# Autodesk Inventor assembly: 200-40-BOGIE-CONNECTOR-ASM-01
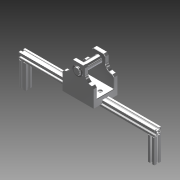
[picture p0: Inventor's stored thumbnail of the model, 180x180]
Saved by Autodesk Inventor 2018.2 (Build 222227000, 227)
## iProperties
Manager: feesmrt
Company: FRANC0R
Created: 2017-12-10
Part Number: 200-40-BOGIE-CONNECTOR-ASM-01
Material: Generisch
Document SubType Name: Assembly
Designer: feesmrt
Project: Rescue Robot
Cost Center: -
Description: Bogie Connector Assembly
Engineer: feesmrt
Authority: feesmrt
Stock Number: 200-40-BOGIE-CONNECTOR-ASM-01
Author: feesmrt
Title: Bogie Connector Assembly
Subject: Rescue Robot
Revision Number: 1
## Documents named in this file (6)
- D:\Programmierung\FRANC0R\CAD\02-Rocker-Bogie-Robot\200-ROCKER-BOGIE\200-40-BOGIE-CONNECTOR-ASM-01.iam
- D:\Programmierung\FRANC0R\CAD\02-Rocker-Bogie-Robot\200-ROCKER-BOGIE\200-40-BOGIE-CONNECTOR-01.ipt
- D:\Programmierung\FRANC0R\CAD\02-Rocker-Bogie-Robot\200-ROCKER-BOGIE\200-40-BOGIE-CONNECTOR-02.ipt
- D:\Programmierung\FRANC0R\CAD\02-Rocker-Bogie-Robot\900-COMPONENTS\900-50-PROFILES\90-50-PROFILES-20x20x400.ipt
- D:\Programmierung\FRANC0R\CAD\02-Rocker-Bogie-Robot\900-COMPONENTS\900-50-PROFILES\90-50-PROFILES-20x20x70.ipt
- D:\Programmierung\FRANC0R\CAD\02-Rocker-Bogie-Robot\900-COMPONENTS\900-60-CIRCLIPS\900-60-CIRCLIPS-DIN6799-15.ipt
## Components (7 placed, 5 different names)
1. 200-40-BOGIE-CONNECTOR-01:1 — Passend:1, Passend:2, Passend:3
2. 200-40-BOGIE-CONNECTOR-02:1 — Passend:1, Passend:6, Passend:7, Passend:8, Passend:9, Passend:12
3. 90-50-PROFILES-20x20x400:1 — Passend:2, Passend:3, Fluchtend:2, Passend:4, Fluchtend:3, Fluchtend:4, Passend:5, Fluchtend:5, Fluchtend:6
4. 90-50-PROFILES-20x20x70:1 — Passend:5, Fluchtend:5, Fluchtend:6
5. 90-50-PROFILES-20x20x70:2 — Passend:4, Fluchtend:3, Fluchtend:4
6. 900-60-CIRCLIPS-DIN6799-15:1 — Passend:6, Passend:7, Passend:10
7. 900-60-CIRCLIPS-DIN6799-15:2 — Passend:8, Passend:9, Passend:11
## Relationships (17: Mate 12, Flush 5)
- Passend:1 [Mate]: 200-40-BOGIE-CONNECTOR-01:1 ↔ 200-40-BOGIE-CONNECTOR-02:1
- Passend:2 [Mate]: 200-40-BOGIE-CONNECTOR-01:1 ↔ 90-50-PROFILES-20x20x400:1
- Passend:3 [Mate]: 200-40-BOGIE-CONNECTOR-01:1 ↔ 90-50-PROFILES-20x20x400:1
- Fluchtend:2 [Flush]: 90-50-PROFILES-20x20x400:1
- Passend:4 [Mate]: 90-50-PROFILES-20x20x400:1 ↔ 90-50-PROFILES-20x20x70:2
- Fluchtend:3 [Flush]: 90-50-PROFILES-20x20x400:1 ↔ 90-50-PROFILES-20x20x70:2
- Fluchtend:4 [Flush]: 90-50-PROFILES-20x20x400:1 ↔ 90-50-PROFILES-20x20x70:2
- Passend:5 [Mate]: 90-50-PROFILES-20x20x400:1 ↔ 90-50-PROFILES-20x20x70:1
- Fluchtend:5 [Flush]: 90-50-PROFILES-20x20x400:1 ↔ 90-50-PROFILES-20x20x70:1
- Fluchtend:6 [Flush]: 90-50-PROFILES-20x20x400:1 ↔ 90-50-PROFILES-20x20x70:1
- Passend:6 [Mate]: 200-40-BOGIE-CONNECTOR-02:1 ↔ 900-60-CIRCLIPS-DIN6799-15:1
- Passend:7 [Mate]: 200-40-BOGIE-CONNECTOR-02:1 ↔ 900-60-CIRCLIPS-DIN6799-15:1
- Passend:8 [Mate]: 200-40-BOGIE-CONNECTOR-02:1 ↔ 900-60-CIRCLIPS-DIN6799-15:2
- Passend:9 [Mate]: 200-40-BOGIE-CONNECTOR-02:1 ↔ 900-60-CIRCLIPS-DIN6799-15:2
- Passend:10 [Mate]: 900-60-CIRCLIPS-DIN6799-15:1
- Passend:11 [Mate]: 900-60-CIRCLIPS-DIN6799-15:2
- Passend:12 [Mate]: 200-40-BOGIE-CONNECTOR-02:1
